# Autodesk Inventor assembly: LeadScrewMotor
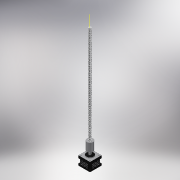
[picture p0: Inventor's stored thumbnail of the model, 180x180]
Saved by Autodesk Inventor 2020 (Build 240168000, 168)
## iProperties
Created: 2018-04-20
Part Number: LeadScrewMotor
Document SubType Name: Assembly
Designer: PC  USER
Author: PC  USER
## Documents named in this file (4)
- C:\Users\pc-konvi\Documents\Lobola\open_source_scrabble\CAD model\LeadScrewMotor.iam
- C:\Users\pc-konvi\Documents\Lobola\open_source_scrabble\CAD model\NEMA14.ipt
- C:\Users\pc-konvi\Documents\Lobola\open_source_scrabble\CAD model\Flx_Al_Coupling(5_8mm).ipt
- C:\Users\pc-konvi\Documents\Lobola\open_source_scrabble\CAD model\TR8x8 lead screw.ipt
## Components (3 placed, 3 different names)
1. NEMA14:1 — Mate:1, Mate:2, Mate:3, Mate:4, Mate:5
2. Flx_Al_Coupling(5_8mm):1 — Mate:4, Mate:5, Mate:6, Flush:1
3. TR8x8 lead screw:1 — Mate:6, Flush:1
## Relationships (7: Mate 6, Flush 1)
- Mate:1: NEMA14:1
- Mate:2: NEMA14:1
- Mate:3: NEMA14:1
- Mate:4: NEMA14:1 ↔ Flx_Al_Coupling(5_8mm):1
- Mate:5: NEMA14:1 ↔ Flx_Al_Coupling(5_8mm):1
- Mate:6: Flx_Al_Coupling(5_8mm):1 ↔ TR8x8 lead screw:1
- Flush:1: Flx_Al_Coupling(5_8mm):1 ↔ TR8x8 lead screw:1
